# Autodesk Inventor assembly: pot arm
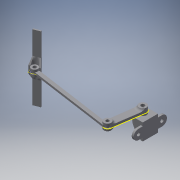
[picture p0: Inventor's stored thumbnail of the model, 180x180]
Saved by Autodesk Inventor 2019 (Build 230136000, 136)
## iProperties
Created: 2019-03-31
Part Number: pot arm
Document SubType Name: Assembly
Designer: torba
Author: torba
## Documents named in this file (5)
- C:\Users\torba\Nextcloud\Projects\Inventor\Plasma 5x10\pot arm.iam
- C:\Users\torba\Nextcloud\Projects\Inventor\Plasma 5x10\POT HOLDER.ipt
- C:\Users\torba\Nextcloud\Projects\Inventor\Plasma 5x10\knuckle.ipt
- C:\Users\torba\Nextcloud\Projects\Inventor\Plasma 5x10\arm.ipt
- C:\Users\torba\Nextcloud\Projects\Inventor\Plasma 5x10\top holder.ipt
## Components (4 placed, 4 different names)
1. POT HOLDER:1 — Mate:1, Mate:2
2. knuckle:1 — Mate:1, Mate:2, Mate:3, Mate:4
3. arm:1 — Mate:3, Mate:4, Mate:5, Mate:6
4. top holder:1 — Mate:5, Mate:6
## Relationships (6: Mate 6)
- Mate:1 (1 mm): POT HOLDER:1 ↔ knuckle:1
- Mate:2: POT HOLDER:1 ↔ knuckle:1
- Mate:3: knuckle:1 ↔ arm:1
- Mate:4: knuckle:1 ↔ arm:1
- Mate:5: arm:1 ↔ top holder:1
- Mate:6: arm:1 ↔ top holder:1
